# Autodesk Inventor assembly: Rail_AssemblyV2_0
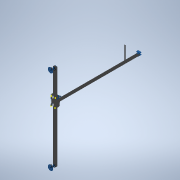
[picture p0: Inventor's stored thumbnail of the model, 180x180]
Saved by Autodesk Inventor 2021 (Build 250183000, 183)
## iProperties
Created: 2021-01-25
Part Number: Rail_AssemblyV2_0
Document SubType Name: Assembly
Designer: Jorian Brusind
Mass: 3786.54 g
Surface Area: 19508.5 cm^2
Volume: 2323.9 cm^3
Density: 1.62939 g/cm^3
Author: Jorian Brusind
## Documents named in this file (31)
- C:\Users\Jorian Brusind\Documents\GitHub\PersonalProjects\HyperRail\Inventor Files\Rail_AssemblyV2_0.iam
- C:\Users\Jorian Brusind\Documents\GitHub\PersonalProjects\Inventor Projects\Useful models\NEMA_Steppers\NEMA23\23HS8430B.ipt
- C:\Users\Jorian Brusind\Documents\GitHub\PersonalProjects\HyperRail\Inventor Files\NEMA23_StepperonlineMount.ipt
- C:\Users\Jorian Brusind\Documents\GitHub\PersonalProjects\Inventor Projects\Useful models\8020_Sets\IPT_20_Series\IPT_20_Series\20-2040_200mm.ipt
- C:\Users\Jorian Brusind\Documents\GitHub\PersonalProjects\HyperRail\Inventor Files\2804S_NEMA2115_1Gearbox.ipt
- C:\Users\Jorian Brusind\Documents\GitHub\PersonalProjects\HyperRail\PCB Files\Integrated Stepper Motor Driver\ExportSTEP\Main.iam
- C:\Users\Jorian Brusind\Documents\GitHub\PersonalProjects\HyperRail\Inventor Files\NEMA23_Shroud.ipt
- C:\Users\Jorian Brusind\Documents\GitHub\PersonalProjects\Inventor Projects\Useful models\8020_Sets\IPT_20_Series\IPT_20_Series\20-4040_2m.ipt
- C:\Users\Jorian Brusind\Documents\GitHub\PersonalProjects\HyperRail\Inventor Files\98952A059_ALUM MALE-FEM THRDED HEX STANDOFF.ipt
- C:\Users\Jorian Brusind\Documents\GitHub\PersonalProjects\HyperRail\Inventor Files\95783A039_NYLON 6-6 MALE-FEM THRDED HEX STANDOFF.ipt
- C:\Users\Jorian Brusind\Documents\GitHub\PersonalProjects\HyperRail\Inventor Files\Integrated_Stepper_NEMA23_Mount.ipt
- C:\Users\Jorian Brusind\Documents\GitHub\PersonalProjects\HyperRail\Inventor Files\Foot_Spacer.ipt
- C:\Users\Jorian Brusind\Documents\GitHub\PersonalProjects\Inventor Projects\Useful models\Metric bolt\Bolt M5 50mm.ipt
- C:\Users\Jorian Brusind\Documents\GitHub\PersonalProjects\Inventor Projects\Useful models\Metric nuts\Nut M5.ipt
- C:\Users\Jorian Brusind\Documents\GitHub\PersonalProjects\HyperRail\Inventor Files\Bottom_Foot.ipt
- C:\Users\Jorian Brusind\Documents\GitHub\PersonalProjects\HyperRail\Inventor Files\90deg_4040Bracket.ipt
- C:\Users\Jorian Brusind\Documents\GitHub\PersonalProjects\HyperRail\Inventor Files\X_Carriage_V2_0.iam
- C:\Users\Jorian Brusind\Documents\GitHub\PersonalProjects\HyperRail\Inventor Files\X_CarriageR_V2_0.iam
- C:\Users\Jorian Brusind\Documents\GitHub\PersonalProjects\Inventor Projects\Useful models\8020_Sets\IPT_40_Series\Extra_40_Series\HFS5-4060-4000\HFS5-4060-2125.ipt
- C:\Users\Jorian Brusind\Documents\GitHub\PersonalProjects\Inventor Projects\Useful models\8020_Sets\IPT_20_Series\IPT_20_Series\20-2040_150mm.ipt
- C:\Users\Jorian Brusind\Documents\GitHub\PersonalProjects\HyperRail\Inventor Files\RightAngle_Bracket_60mm.ipt
- C:\Users\Jorian Brusind\Documents\GitHub\PersonalProjects\HyperRail\Inventor Files\X_CarriageR_V2_0_Short.iam
- C:\Users\Jorian Brusind\Documents\GitHub\PersonalProjects\HyperRail\Inventor Files\X_CarriageL_V2_0_Short.iam
- C:\Users\Jorian Brusind\Documents\GitHub\PersonalProjects\Inventor Projects\Useful models\e2-micro-e-chains-small-and-lightweight-e-chains\03_07_012_0_160_5.iam
- C:\Users\Jorian Brusind\Documents\GitHub\PersonalProjects\HyperRail\Inventor Files\Cable_Guide_End.ipt
- C:\Users\Jorian Brusind\Documents\GitHub\PersonalProjects\HyperRail\Inventor Files\Belt_Clamp.ipt
- C:\Users\Jorian Brusind\Documents\GitHub\PersonalProjects\HyperRail\Inventor Files\SmallBelt_LargePulley_70mm.ipt
- C:\Users\Jorian Brusind\Documents\GitHub\PersonalProjects\Inventor Projects\Useful models\8020_Sets\AIS2018\20-2568_d.iam
- C:\Users\Jorian Brusind\Documents\GitHub\PersonalProjects\HyperRail\Inventor Files\5mm_bore_10mm_width_idlepulley.ipt
- C:\Users\Jorian Brusind\Documents\GitHub\PersonalProjects\HyperRail\Inventor Files\Idler_Spacer.ipt
- C:\Users\Jorian Brusind\Documents\GitHub\PersonalProjects\HyperRail\Inventor Files\Tape_Belt_Layer.ipt
## Components (46 placed, 30 different names)
1. 23HS8430B:1 — Mate:127, Angle:3, Mate:158, Mate:177, Mate:179, Mate:180, Mate:181, Mate:182, Mate:183, Mate:184, Mate:185, Mate:264, Mate:265, Mate:295
2. NEMA23_StepperonlineMount:1 — Angle:2, Mate:98, Mate:128, Mate:289, Flush:99, Mate:303, Mate:304, Flush:107, Flush:108
3. 20-2040_200mm:1 — Mate:253, Flush:83, Flush:84, Flush:88, Mate:284, Mate:297, Mate:301, Mate:302, Flush:111, Flush:112
4. 2804S_NEMA2115_1Gearbox:1 — Angle:2, Mate:98, Mate:127, Mate:128, Angle:3, Mate:158, Flush:86, Mate:321, Flush:122
5. Main:1 [sub-assembly] — Mate:291, Mate:292, Mate:293
6. 20-4040_2m:2 — Mate:232, Flush:73, Mate:233, Mate:234, Flush:74, Mate:288, Flush:98, Flush:123, Mate:322, Mate:323, Mate:326, Mate:327, Mate:330, Mate:331, Flush:124
7. NEMA23_Shroud:1 — Mate:264, Mate:265, Flush:86, Mate:294
8. 98952A059_ALUM MALE-FEM THRDED HEX STANDOFF:1 — Mate:180, Mate:181, Mate:186, Mate:191
9. 98952A059_ALUM MALE-FEM THRDED HEX STANDOFF:2 — Mate:184, Mate:185, Mate:189, Mate:192
10. 98952A059_ALUM MALE-FEM THRDED HEX STANDOFF:3 — Mate:177, Mate:179, Mate:187, Mate:190
11. 98952A059_ALUM MALE-FEM THRDED HEX STANDOFF:4 — Mate:182, Mate:183, Mate:188, Mate:193
12. 95783A039_NYLON 6-6 MALE-FEM THRDED HEX STANDOFF:1 — Mate:188, Mate:193
13. 95783A039_NYLON 6-6 MALE-FEM THRDED HEX STANDOFF:2 — Mate:186, Mate:191
14. 95783A039_NYLON 6-6 MALE-FEM THRDED HEX STANDOFF:3 — Mate:187, Mate:190
15. 95783A039_NYLON 6-6 MALE-FEM THRDED HEX STANDOFF:4 — Mate:189, Mate:192
16. Bolt M5 50mm:1 — Mate:224, Mate:245, Mate:246, Mate:247, Mate:269
17. Nut M5:1 — Mate:226, Mate:247
18. Nut M5:2 — Mate:244, Flush:78, Mate:246
19. Bottom_Foot:1 — Mate:224, Mate:226, Mate:245, Flush:81, Flush:93
20. 90deg_4040Bracket:1 — Mate:232, Flush:73, Mate:233, Flush:75
21. 90deg_4040Bracket:2 — Mate:234, Flush:74, Flush:75
22. Foot_Spacer:1 — Mate:244, Flush:78, Mate:269, Mate:283, Flush:94
23. Foot_Spacer:2 — Mate:250, Mate:281, Flush:91, Flush:92, Mate:282
24. Bottom_Foot:2 — Mate:249, Mate:251, Flush:81, Flush:93
25. Bolt M5 50mm:2 — Mate:249, Mate:250, Mate:251, Mate:282
26. X_Carriage_V2_0:1 [sub-assembly] — Mate:253, Flush:83, Flush:84, Flush:113, Mate:319
27. 20-2040_200mm:2 — Flush:88, Mate:286, Flush:96, Mate:305, Flush:111, Mate:312, Flush:114, Flush:116, Mate:316, Flush:117, Flush:124
28. HFS5-4060-2125:1 — Mate:277, Mate:278, Mate:279, Mate:280, Mate:281, Flush:91, Flush:92, Mate:283, Flush:94, Mate:284, Flush:114, Mate:313, Flush:115, Mate:317, Flush:118, Flush:119, Flush:120, Mate:318, Flush:121, Mate:332, Mate:333
29. 20-2040_150mm:1 — Mate:286, Flush:96, Mate:288, Flush:98, Mate:289, Flush:99, Mate:310
30. Integrated_Stepper_NEMA23_Mount:1 — Mate:291, Mate:292, Mate:293, Mate:294, Mate:295
31. X_CarriageR_V2_0:2 [sub-assembly] — Mate:297, Flush:112, Flush:113, Mate:311
32. RightAngle_Bracket_60mm:1 — Mate:301, Mate:304, Flush:107
33. RightAngle_Bracket_60mm:2 — Mate:302, Mate:303, Flush:108
34. X_CarriageR_V2_0_Short:1 [sub-assembly] — Mate:305, Mate:310, Mate:319
35. X_CarriageL_V2_0_Short:1 [sub-assembly] — Mate:311, Mate:312
36. 03_07_012_0_160_5:1 [sub-assembly] — Mate:313, Flush:115, Mate:320
37. Cable_Guide_End:1 — Flush:116, Mate:316, Flush:117, Mate:320
38. Belt_Clamp:1 — Mate:317, Flush:118, Flush:119
39. Belt_Clamp:2 — Flush:120, Mate:318, Flush:121
40. SmallBelt_LargePulley_70mm:1 — Mate:321, Flush:122
41. 20-2568_d:1 [sub-assembly] — Flush:123, Mate:322, Mate:323
42. 5mm_bore_10mm_width_idlepulley:1 — Mate:324, Mate:325, Angle:4
43. Idler_Spacer:1 — Mate:324, Mate:325, Mate:326, Mate:327
44. 5mm_bore_10mm_width_idlepulley:2 — Mate:328, Mate:329, Angle:4
45. Idler_Spacer:2 — Mate:328, Mate:329, Mate:330, Mate:331
46. Tape_Belt_Layer:1 — Mate:332, Mate:333
## Relationships (115: Mate 80, Flush 32, Angle 3)
- Angle:2 (0 deg): NEMA23_StepperonlineMount:1 ↔ 2804S_NEMA2115_1Gearbox:1
- Mate:98: NEMA23_StepperonlineMount:1 ↔ 2804S_NEMA2115_1Gearbox:1
- Mate:127: 23HS8430B:1 ↔ 2804S_NEMA2115_1Gearbox:1
- Mate:128: NEMA23_StepperonlineMount:1 ↔ 2804S_NEMA2115_1Gearbox:1
- Angle:3 (0 deg): 23HS8430B:1 ↔ 2804S_NEMA2115_1Gearbox:1
- Mate:158: 23HS8430B:1 ↔ 2804S_NEMA2115_1Gearbox:1
- Mate:177: 23HS8430B:1 ↔ 98952A059_ALUM MALE-FEM THRDED HEX STANDOFF:3
- Mate:179: 23HS8430B:1 ↔ 98952A059_ALUM MALE-FEM THRDED HEX STANDOFF:3
- Mate:180: 23HS8430B:1 ↔ 98952A059_ALUM MALE-FEM THRDED HEX STANDOFF:1
- Mate:181: 23HS8430B:1 ↔ 98952A059_ALUM MALE-FEM THRDED HEX STANDOFF:1
- Mate:182: 23HS8430B:1 ↔ 98952A059_ALUM MALE-FEM THRDED HEX STANDOFF:4
- Mate:183: 23HS8430B:1 ↔ 98952A059_ALUM MALE-FEM THRDED HEX STANDOFF:4
- Mate:184: 23HS8430B:1 ↔ 98952A059_ALUM MALE-FEM THRDED HEX STANDOFF:2
- Mate:185: 23HS8430B:1 ↔ 98952A059_ALUM MALE-FEM THRDED HEX STANDOFF:2
- Mate:186: 98952A059_ALUM MALE-FEM THRDED HEX STANDOFF:1 ↔ 95783A039_NYLON 6-6 MALE-FEM THRDED HEX STANDOFF:2
- Mate:187: 98952A059_ALUM MALE-FEM THRDED HEX STANDOFF:3 ↔ 95783A039_NYLON 6-6 MALE-FEM THRDED HEX STANDOFF:3
- Mate:188: 98952A059_ALUM MALE-FEM THRDED HEX STANDOFF:4 ↔ 95783A039_NYLON 6-6 MALE-FEM THRDED HEX STANDOFF:1
- Mate:189: 98952A059_ALUM MALE-FEM THRDED HEX STANDOFF:2 ↔ 95783A039_NYLON 6-6 MALE-FEM THRDED HEX STANDOFF:4
- Mate:190: 98952A059_ALUM MALE-FEM THRDED HEX STANDOFF:3 ↔ 95783A039_NYLON 6-6 MALE-FEM THRDED HEX STANDOFF:3
- Mate:191: 98952A059_ALUM MALE-FEM THRDED HEX STANDOFF:1 ↔ 95783A039_NYLON 6-6 MALE-FEM THRDED HEX STANDOFF:2
- Mate:192: 98952A059_ALUM MALE-FEM THRDED HEX STANDOFF:2 ↔ 95783A039_NYLON 6-6 MALE-FEM THRDED HEX STANDOFF:4
- Mate:193: 98952A059_ALUM MALE-FEM THRDED HEX STANDOFF:4 ↔ 95783A039_NYLON 6-6 MALE-FEM THRDED HEX STANDOFF:1
- Mate:224: Bolt M5 50mm:1 ↔ Bottom_Foot:1
- Mate:226: Nut M5:1 ↔ Bottom_Foot:1
- Mate:232: 20-4040_2m:2 ↔ 90deg_4040Bracket:1
- Flush:73: 20-4040_2m:2 ↔ 90deg_4040Bracket:1
- Mate:233: 20-4040_2m:2 ↔ 90deg_4040Bracket:1
- Mate:234: 20-4040_2m:2 ↔ 90deg_4040Bracket:2
- Flush:74: 20-4040_2m:2 ↔ 90deg_4040Bracket:2
- Flush:75: 90deg_4040Bracket:1 ↔ 90deg_4040Bracket:2
- Mate:244: Nut M5:2 ↔ Foot_Spacer:1
- Flush:78: Nut M5:2 ↔ Foot_Spacer:1
- Mate:245: Bolt M5 50mm:1 ↔ Bottom_Foot:1
- Mate:246: Bolt M5 50mm:1 ↔ Nut M5:2
- Mate:247: Bolt M5 50mm:1 ↔ Nut M5:1
- Mate:249: Bottom_Foot:2 ↔ Bolt M5 50mm:2
- Mate:250: Foot_Spacer:2 ↔ Bolt M5 50mm:2
- Mate:251: Bottom_Foot:2 ↔ Bolt M5 50mm:2
- Flush:81: Bottom_Foot:1 ↔ Bottom_Foot:2
- Mate:253: 20-2040_200mm:1 ↔ X_Carriage_V2_0:1
- Flush:83 (-30.5 mm): 20-2040_200mm:1 ↔ X_Carriage_V2_0:1
- Flush:84 (-10 mm): 20-2040_200mm:1 ↔ X_Carriage_V2_0:1
- Mate:264 (1 mm): 23HS8430B:1 ↔ NEMA23_Shroud:1
- Mate:265 (1 mm): 23HS8430B:1 ↔ NEMA23_Shroud:1
- Mate:269: Bolt M5 50mm:1 ↔ Foot_Spacer:1
- Flush:86: 2804S_NEMA2115_1Gearbox:1 ↔ NEMA23_Shroud:1
- Flush:88: 20-2040_200mm:1 ↔ 20-2040_200mm:2
- Mate:277: HFS5-4060-2125:1
- Mate:278: HFS5-4060-2125:1
- Mate:279: HFS5-4060-2125:1
- Mate:280: HFS5-4060-2125:1
- Mate:281: Foot_Spacer:2 ↔ HFS5-4060-2125:1
- Flush:91: Foot_Spacer:2 ↔ HFS5-4060-2125:1
- Flush:92 (20 mm): Foot_Spacer:2 ↔ HFS5-4060-2125:1
- Mate:282: Foot_Spacer:2 ↔ Bolt M5 50mm:2
- Flush:93: Bottom_Foot:1 ↔ Bottom_Foot:2
- Mate:283 (-40 mm): Foot_Spacer:1 ↔ HFS5-4060-2125:1
- Flush:94: Foot_Spacer:1 ↔ HFS5-4060-2125:1
- Mate:284 (24 mm): 20-2040_200mm:1 ↔ HFS5-4060-2125:1
- Mate:286: 20-2040_200mm:2 ↔ 20-2040_150mm:1
- Flush:96 (-5 mm): 20-2040_200mm:2 ↔ 20-2040_150mm:1
- Mate:288: 20-4040_2m:2 ↔ 20-2040_150mm:1
- Flush:98: 20-4040_2m:2 ↔ 20-2040_150mm:1
- Mate:289 (10 mm): NEMA23_StepperonlineMount:1 ↔ 20-2040_150mm:1
- Flush:99 (-12.5 mm): NEMA23_StepperonlineMount:1 ↔ 20-2040_150mm:1
- Mate:291: Main:1 ↔ Integrated_Stepper_NEMA23_Mount:1
- Mate:292: Main:1 ↔ Integrated_Stepper_NEMA23_Mount:1
- Mate:293: Main:1 ↔ Integrated_Stepper_NEMA23_Mount:1
- Mate:294: NEMA23_Shroud:1 ↔ Integrated_Stepper_NEMA23_Mount:1
- Mate:295: 23HS8430B:1 ↔ Integrated_Stepper_NEMA23_Mount:1
- Mate:297: 20-2040_200mm:1 ↔ X_CarriageR_V2_0:2
- Mate:301: 20-2040_200mm:1 ↔ RightAngle_Bracket_60mm:1
- Mate:302: 20-2040_200mm:1 ↔ RightAngle_Bracket_60mm:2
- Mate:303: NEMA23_StepperonlineMount:1 ↔ RightAngle_Bracket_60mm:2
- Mate:304: NEMA23_StepperonlineMount:1 ↔ RightAngle_Bracket_60mm:1
- Flush:107: NEMA23_StepperonlineMount:1 ↔ RightAngle_Bracket_60mm:1
- Flush:108: NEMA23_StepperonlineMount:1 ↔ RightAngle_Bracket_60mm:2
- Mate:305: 20-2040_200mm:2 ↔ X_CarriageR_V2_0_Short:1
- Flush:111: 20-2040_200mm:1 ↔ 20-2040_200mm:2
- Mate:310 (15 mm): 20-2040_150mm:1 ↔ X_CarriageR_V2_0_Short:1
- Flush:112 (-10 mm): 20-2040_200mm:1 ↔ X_CarriageR_V2_0:2
- Flush:113: X_Carriage_V2_0:1 ↔ X_CarriageR_V2_0:2
- Mate:311: X_CarriageR_V2_0:2 ↔ X_CarriageL_V2_0_Short:1
- Mate:312: 20-2040_200mm:2 ↔ X_CarriageL_V2_0_Short:1
- Flush:114: 20-2040_200mm:2 ↔ HFS5-4060-2125:1
- Mate:313 (2 mm): HFS5-4060-2125:1 ↔ 03_07_012_0_160_5:1
- Flush:115: HFS5-4060-2125:1 ↔ 03_07_012_0_160_5:1
- Flush:116: 20-2040_200mm:2 ↔ Cable_Guide_End:1
- Mate:316: 20-2040_200mm:2 ↔ Cable_Guide_End:1
- Flush:117: 20-2040_200mm:2 ↔ Cable_Guide_End:1
- Mate:317: HFS5-4060-2125:1 ↔ Belt_Clamp:1
- Flush:118: HFS5-4060-2125:1 ↔ Belt_Clamp:1
- Flush:119: HFS5-4060-2125:1 ↔ Belt_Clamp:1
- Flush:120: HFS5-4060-2125:1 ↔ Belt_Clamp:2
- Mate:318: HFS5-4060-2125:1 ↔ Belt_Clamp:2
- Flush:121: HFS5-4060-2125:1 ↔ Belt_Clamp:2
- Mate:319: X_Carriage_V2_0:1 ↔ X_CarriageR_V2_0_Short:1
- Mate:320: 03_07_012_0_160_5:1 ↔ Cable_Guide_End:1
- Mate:321: 2804S_NEMA2115_1Gearbox:1 ↔ SmallBelt_LargePulley_70mm:1
- Flush:122 (3 mm): 2804S_NEMA2115_1Gearbox:1 ↔ SmallBelt_LargePulley_70mm:1
- Flush:123: 20-4040_2m:2 ↔ 20-2568_d:1
- Mate:322 (-2 mm): 20-4040_2m:2 ↔ 20-2568_d:1
- Mate:323: 20-4040_2m:2 ↔ 20-2568_d:1
- Mate:324: 5mm_bore_10mm_width_idlepulley:1 ↔ Idler_Spacer:1
- Mate:325: 5mm_bore_10mm_width_idlepulley:1 ↔ Idler_Spacer:1
- Mate:326: 20-4040_2m:2 ↔ Idler_Spacer:1
- Mate:327 (2.5 mm): 20-4040_2m:2 ↔ Idler_Spacer:1
- Mate:328: 5mm_bore_10mm_width_idlepulley:2 ↔ Idler_Spacer:2
- Mate:329: 5mm_bore_10mm_width_idlepulley:2 ↔ Idler_Spacer:2
- Mate:330 (15 mm): 20-4040_2m:2 ↔ Idler_Spacer:2
- Mate:331 (2.5 mm): 20-4040_2m:2 ↔ Idler_Spacer:2
- Angle:4 (0 deg): 5mm_bore_10mm_width_idlepulley:1 ↔ 5mm_bore_10mm_width_idlepulley:2
- Flush:124 (20 mm): 20-4040_2m:2 ↔ 20-2040_200mm:2
- Mate:332: HFS5-4060-2125:1 ↔ Tape_Belt_Layer:1
- Mate:333 (1 mm): HFS5-4060-2125:1 ↔ Tape_Belt_Layer:1
